# Autodesk Inventor assembly: 8-mm lead screw
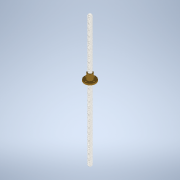
[picture p0: Inventor's stored thumbnail of the model, 180x180]
Saved by Autodesk Inventor 2020 (Build 240168000, 168)
## iProperties
Created: 2022-09-10
Part Number: 8-mm lead screw
Document SubType Name: Assembly
Designer: Andrew
Author: Andrew
## Documents named in this file (3)
- C:\Users\Andrew\Documents\Works\CAD\Inventor\Lead Screw\8-mm lead screw.iam
- C:\Users\Andrew\Documents\Works\CAD\Inventor\Lead Screw\Lead Screw.ipt
- C:\Users\Andrew\Documents\Works\CAD\Inventor\Lead Screw\Nut.ipt
## Components (2 placed, 2 different names)
1. Lead Screw:1 — Mate:1, Mate:2, Mate:3, Flush:1
2. Nut:1 — Mate:3, Flush:1
## Relationships (4: Mate 3, Flush 1)
- Mate:1: Lead Screw:1
- Mate:2: Lead Screw:1
- Mate:3: Lead Screw:1 ↔ Nut:1
- Flush:1: Lead Screw:1 ↔ Nut:1
